# Autodesk Inventor assembly: Montagem_Drone1
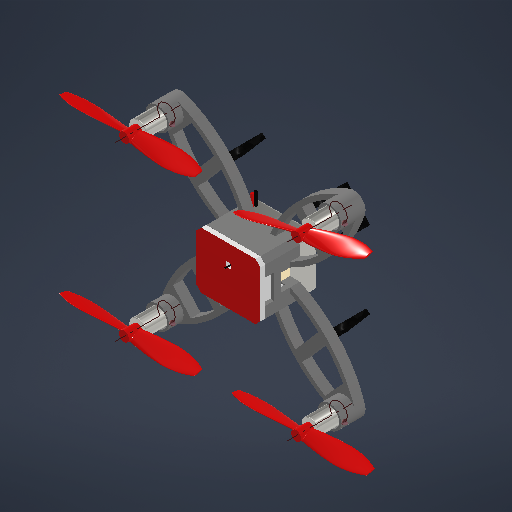
[picture p0: Inventor's stored thumbnail of the model, 512x512]
Saved by Autodesk Inventor 2027 (Build 310192000, 192)
## iProperties
Created: 2026-07-17
Part Number: Montagem_Drone1
Document SubType Name: Assembly
Designer: marcu
Mass: 19.2027 g
Surface Area: 228.132 cm^2
Volume: 19.2027 cm^3
Density: 1 g/cm^3
Author: marcu
## Documents named in this file (8)
- C:\Users\marcu\projetos\cin-maker\Projeto_drone\Montagem_Drone1.iam
- C:\Users\marcu\projetos\cin-maker\Projeto_drone\Frame1.ipt
- C:\Users\marcu\projetos\cin-maker\Projeto_drone\Placas_Eletrônicas.iam
- Placas_Eletrônicas.iam
- C:\Users\marcu\projetos\cin-maker\Projeto_drone\Bateria.ipt
- C:\Users\marcu\projetos\cin-maker\Projeto_drone\Trem_Pouso.ipt
- C:\Users\marcu\projetos\cin-maker\Projeto_drone\TampaEletronica.ipt
- C:\Users\marcu\projetos\cin-maker\Projeto_drone\Unidade_de_potência.iam
## Components (12 placed, 6 different names)
1. Frame1:1 — Coincidente:1, Coincidente:2, Coincidente:3, Coincidente:4, Coincidente:5, Coincidente:6, Coincidente:7, Coincidente:8, Coincidente:9, Coincidente:10, Coincidente:11, Coincidente:12, Coincidente:13, Coincidente:18, Coincidente:19, Coincidente:20, Coincidente:21, Coincidente:22, Coincidente:23, Coincidente:24, Coincidente:25, Coincidente:26, Coincidente:27, Coincidente:28, Coincidente:29, Coincidente:30, Coincidente:31, Coincidente:32, Coincidente:33, Coincidente:34
2. Placas_Eletrônicas:1 [sub-assembly] — Coincidente:20, Coincidente:21, Coincidente:22
3. Bateria:1 — Coincidente:33, Coincidente:34, Coincidente:35
4. Trem_Pouso:1 — Coincidente:11, Coincidente:12, Coincidente:13
5. Trem_Pouso:2 — Coincidente:8, Coincidente:9, Coincidente:10, Coincidente:35
6. Trem_Pouso:3 — Coincidente:5, Coincidente:6, Coincidente:7
7. Trem_Pouso:4 — Coincidente:1, Coincidente:2, Coincidente:3, Coincidente:4
8. TampaEletronica:1 — Coincidente:18, Coincidente:19, Coincidente:23
9. Unidade_de_potência:1 [sub-assembly] — Coincidente:24, Coincidente:25
10. Unidade_de_potência:2 [sub-assembly] — Coincidente:26, Coincidente:27
11. Unidade_de_potência:3 [sub-assembly] — Coincidente:28, Coincidente:29
12. Unidade_de_potência:4 [sub-assembly] — Coincidente:30, Coincidente:31
## Relationships (31: Mate 31)
- Coincidente:1 [Mate]: Frame1:1 ↔ Trem_Pouso:4
- Coincidente:2 [Mate]: Frame1:1 ↔ Trem_Pouso:4
- Coincidente:3 [Mate]: Frame1:1 ↔ Trem_Pouso:4
- Coincidente:4 [Mate]: Frame1:1 ↔ Trem_Pouso:4
- Coincidente:5 [Mate]: Frame1:1 ↔ Trem_Pouso:3
- Coincidente:6 [Mate]: Frame1:1 ↔ Trem_Pouso:3
- Coincidente:7 [Mate]: Frame1:1 ↔ Trem_Pouso:3
- Coincidente:8 [Mate]: Frame1:1 ↔ Trem_Pouso:2
- Coincidente:9 [Mate]: Frame1:1 ↔ Trem_Pouso:2
- Coincidente:10 [Mate]: Frame1:1 ↔ Trem_Pouso:2
- Coincidente:11 [Mate]: Frame1:1 ↔ Trem_Pouso:1
- Coincidente:12 [Mate]: Frame1:1 ↔ Trem_Pouso:1
- Coincidente:13 [Mate]: Frame1:1 ↔ Trem_Pouso:1
- Coincidente:18 [Mate] (0.2 mm): Frame1:1 ↔ TampaEletronica:1
- Coincidente:19 [Mate] (0.2 mm): Frame1:1 ↔ TampaEletronica:1
- Coincidente:20 [Mate] (1.5 mm): Frame1:1 ↔ Placas_Eletrônicas:1
- Coincidente:21 [Mate]: Frame1:1 ↔ Placas_Eletrônicas:1
- Coincidente:22 [Mate]: Frame1:1 ↔ Placas_Eletrônicas:1
- Coincidente:23 [Mate]: Frame1:1 ↔ TampaEletronica:1
- Coincidente:24 [Mate]: Frame1:1 ↔ Unidade_de_potência:1
- Coincidente:25 [Mate]: Frame1:1 ↔ Unidade_de_potência:1
- Coincidente:26 [Mate]: Frame1:1 ↔ Unidade_de_potência:2
- Coincidente:27 [Mate]: Frame1:1 ↔ Unidade_de_potência:2
- Coincidente:28 [Mate]: Frame1:1 ↔ Unidade_de_potência:3
- Coincidente:29 [Mate]: Frame1:1 ↔ Unidade_de_potência:3
- Coincidente:30 [Mate]: Frame1:1 ↔ Unidade_de_potência:4
- Coincidente:31 [Mate]: Frame1:1 ↔ Unidade_de_potência:4
- Coincidente:32 [Mate]: Frame1:1
- Coincidente:33 [Mate]: Frame1:1 ↔ Bateria:1
- Coincidente:34 [Mate] (0.5 mm): Frame1:1 ↔ Bateria:1
- Coincidente:35 [Mate] (11 mm): Bateria:1 ↔ Trem_Pouso:2
## Named parameters: Finish10_Area = 0.0019635, Finish10_Thickness = 0.008 mm, Finish11_Area = 0.228983, Finish11_Thickness = 0.008 mm, Finish12_Area = 102.659, Finish12_Thickness = 0.008 mm, Finish1_Area = 15.7729, Finish1_Thickness = 0.008 mm, Finish2_Area = 0.199805, Finish2_Thickness = 0.008 mm, Finish3_Area = 0.199805, Finish3_Thickness = 0.008 mm, Finish4_Area = 14.1412, Finish4_Thickness = 0.008 mm, Finish5_Area = 0.00214602, Finish5_Thickness = 0.008 mm, Finish6_Area = 8.68127, Finish6_Thickness = 0.008 mm, Finish7_Area = 2.21, Finish7_Thickness = 0.008 mm, Finish8_Area = 0.228983, Finish8_Thickness = 0.008 mm, Finish9_Area = 0.0019635, Finish9_Thickness = 0.008 mm
note: some values were not read from the file. Shown as the stored number, unit unknown: "Finish10_Area", "Finish11_Area", "Finish12_Area", "Finish1_Area", "Finish2_Area", "Finish3_Area", "Finish4_Area", "Finish5_Area", "Finish6_Area", "Finish7_Area", "Finish8_Area", "Finish9_Area".
